# Autodesk Inventor assembly: 9gServeFrontWheel
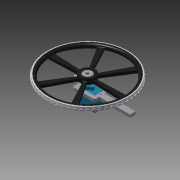
[picture p0: Inventor's stored thumbnail of the model, 180x180]
Saved by Autodesk Inventor 2014 SP1 (Build 180222100, 222)
## iProperties
Created: 2017-01-16
Part Number: 9gServeFrontWheel
Document SubType Name: Assembly
Designer: danielsikar
Author: danielsikar
## Documents named in this file (4)
- C:\Users\danielsikar\Documents\Inventor\IoT-Trike\Assemblies\9gServeFrontWheel.iam
- C:\Users\danielsikar\Documents\Inventor\IoT-Trike\Assemblies\ServoAndBlade.iam
- C:\Users\danielsikar\Documents\Inventor\IoT-Trike\Assemblies\WheelTyre624Bearing.iam
- C:\Users\danielsikar\Documents\Inventor\IoT-Trike\Assemblies\Fork.ipt
## Components (3 placed, 3 different names)
1. ServoAndBlade:1 [sub-assembly] — Mate:1, Mate:2, Mate:3, Mate:4, Mate:5, Flush:1
2. WheelTyre624Bearing:1 [sub-assembly] — Mate:4, Mate:5
3. Fork:1 — Flush:1
## Relationships (6: Mate 5, Flush 1)
- Mate:1: ServoAndBlade:1
- Mate:2: ServoAndBlade:1
- Mate:3: ServoAndBlade:1
- Mate:4: ServoAndBlade:1 ↔ WheelTyre624Bearing:1
- Mate:5 (1 mm): ServoAndBlade:1 ↔ WheelTyre624Bearing:1
- Flush:1: ServoAndBlade:1 ↔ Fork:1
